# Autodesk Inventor assembly: V3IntakeNEW
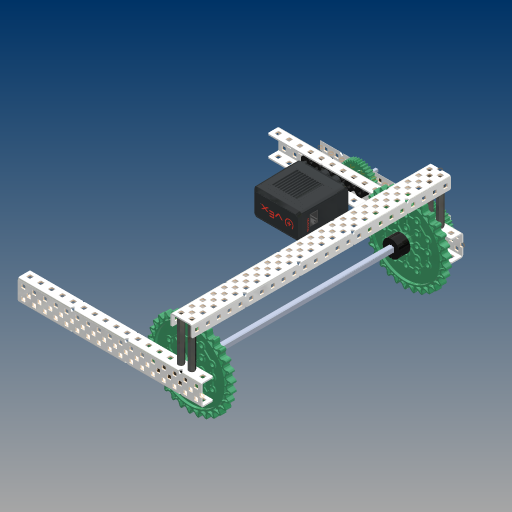
[picture p0: Inventor's stored thumbnail of the model, 512x512]
Saved by Autodesk Inventor 2024 (Build 280153000, 153)
## iProperties
Created: 2023-09-16
Part Number: V3IntakeNEW
Document SubType Name: Assembly
Designer: eddie
Author: eddie
## Documents named in this file (18)
- C:\Users\eddie\Documents\81208X-Over-Under-CAD\V3\V3IntakeNEW.iam
- C:\Users\eddie\Documents\81208X-Over-Under-CAD\VEX-CAD-Inventor-1.4.0\Structure\C Channel\Aluminum 1x2x1\Alu C 1x2x1x17.ipt
- C:\Users\eddie\Documents\81208X-Over-Under-CAD\VEX-CAD-Inventor-1.4.0\Structure\Standoff\Standoff 2.00.ipt
- C:\Users\eddie\Documents\81208X-Over-Under-CAD\VEX-CAD-Inventor-1.4.0\Structure\Standoff.ipt
- C:\Users\eddie\Documents\81208X-Over-Under-CAD\VEX-CAD-Inventor-1.4.0\Structure\C Channel\Aluminum 1x2x1\Alu C 1x2x1x24.ipt
- C:\Users\eddie\Documents\81208X-Over-Under-CAD\VEX-CAD-Inventor-1.4.0\Motion\Shaft LS\Bearing Flat.ipt
- C:\Users\eddie\Documents\81208X-Over-Under-CAD\VEX-CAD-Inventor-1.4.0\Motion\Spacers\Spacer Nylon .375 OD\NSpacer .375 OD x .500.ipt
- C:\Users\eddie\Documents\81208X-Over-Under-CAD\VEX-CAD-Inventor-1.4.0\Motion\Spacers\Spacer Nylon .375 OD.ipt
- C:\Users\eddie\Documents\81208X-Over-Under-CAD\VEX-CAD-Inventor-1.4.0\Motion\Shaft HS\Shaft HS\Shaft HS 12.0 in.ipt
- C:\Users\eddie\Documents\81208X-Over-Under-CAD\VEX-CAD-Inventor-1.4.0\Motion\Shaft HS\Shaft HS.ipt
- C:\Users\eddie\Documents\81208X-Over-Under-CAD\VEX-CAD-Inventor-1.4.0\Motion\Sprockets\9P Sprocket\9P 30T Sprocket, No Insert.iam
- C:\Users\eddie\Documents\81208X-Over-Under-CAD\VEX-CAD-Inventor-1.4.0\Motion\Sprockets\9P Sprocket.iam
- C:\Users\eddie\Documents\81208X-Over-Under-CAD\VEX-CAD-Inventor-1.4.0\Motion\Shaft HS\HS Shaft Collar.ipt
- C:\Users\eddie\Documents\81208X-Over-Under-CAD\VEX-CAD-Inventor-1.4.0\Motion\Gears\LS 36T Gear.ipt
- C:\Users\eddie\Documents\81208X-Over-Under-CAD\Custom-parts\2x12 c channel no sides.ipt
- C:\Users\eddie\Documents\81208X-Over-Under-CAD\VEX-CAD-Inventor-1.4.0\Motion\Shaft LS\Shaft LS.ipt
- C:\Users\eddie\Documents\81208X-Over-Under-CAD\VEX-CAD-Inventor-1.4.0\Motion\Shaft LS\Shaft LS\Shaft LS 1.0.ipt
- C:\Users\eddie\Documents\81208X-Over-Under-CAD\VEX-CAD-Inventor-1.4.0\Electronics\V5 Motor.ipt
## Components (24 placed, 12 different names)
1. Alu C 1x2x1x17:1 — Insert:1, Insert:2, Insert:7
2. Alu C 1x2x1x17:2 — Insert:4, Insert:5, Insert:10, Insert:16, Insert:21, Insert:22, Insert:23, Insert:24
3. Standoff 2.00:1 — Insert:2
4. Standoff 2.00:2 — Insert:1, Insert:3
5. Alu C 1x2x1x24:1 — Insert:3, Insert:6
6. Standoff 2.00:3 — Insert:5, Insert:6
7. Standoff 2.00:4 — Insert:4
8. Bearing Flat:1 — Insert:7, Insert:8, Insert:9
9. NSpacer .375 OD x .500:1 — Insert:8, Insert:12
10. Shaft HS 12.0 in:1 — Insert:9
11. Bearing Flat:2 — Insert:10, Insert:11
12. NSpacer .375 OD x .500:2 — Insert:11, Insert:13
13. 9P 30T Sprocket, No Insert:1 [sub-assembly] — Insert:12, Insert:14
14. 9P 30T Sprocket, No Insert:2 [sub-assembly] — Insert:13, Insert:26
15. HS Shaft Collar:1 — Insert:14
16. LS 36T Gear:1 — Insert:16, Insert:19
17. 2x12 c channel no sides:1 — Insert:19, Insert:20
18. Bearing Flat:3 — Insert:20
19. Shaft LS 1.0:1 — Insert:21
20. LS 36T Gear:2 — Insert:22
21. Bearing Flat:4 — Insert:23
22. Bearing Flat:5 — Insert:24, Insert:25
23. V5 Motor:1 — Insert:25
24. HS Shaft Collar:3 — Insert:26
## Relationships (23: Insert 23)
- Insert:1: Alu C 1x2x1x17:1 ↔ Standoff 2.00:2
- Insert:2: Alu C 1x2x1x17:1 ↔ Standoff 2.00:1
- Insert:3: Standoff 2.00:2 ↔ Alu C 1x2x1x24:1
- Insert:4: Alu C 1x2x1x17:2 ↔ Standoff 2.00:4
- Insert:5: Alu C 1x2x1x17:2 ↔ Standoff 2.00:3
- Insert:6: Alu C 1x2x1x24:1 ↔ Standoff 2.00:3
- Insert:7: Alu C 1x2x1x17:1 ↔ Bearing Flat:1
- Insert:8: Bearing Flat:1 ↔ NSpacer .375 OD x .500:1
- Insert:9: Bearing Flat:1 ↔ Shaft HS 12.0 in:1
- Insert:10: Alu C 1x2x1x17:2 ↔ Bearing Flat:2
- Insert:11: Bearing Flat:2 ↔ NSpacer .375 OD x .500:2
- Insert:12: NSpacer .375 OD x .500:1 ↔ 9P 30T Sprocket, No Insert:1
- Insert:13: NSpacer .375 OD x .500:2 ↔ 9P 30T Sprocket, No Insert:2
- Insert:14: 9P 30T Sprocket, No Insert:1 ↔ HS Shaft Collar:1
- Insert:16: Alu C 1x2x1x17:2 ↔ LS 36T Gear:1
- Insert:19: LS 36T Gear:1 ↔ 2x12 c channel no sides:1
- Insert:20: 2x12 c channel no sides:1 ↔ Bearing Flat:3
- Insert:21: Alu C 1x2x1x17:2 ↔ Shaft LS 1.0:1
- Insert:22: Alu C 1x2x1x17:2 ↔ LS 36T Gear:2
- Insert:23: Alu C 1x2x1x17:2 ↔ Bearing Flat:4
- Insert:24: Alu C 1x2x1x17:2 ↔ Bearing Flat:5
- Insert:25: Bearing Flat:5 ↔ V5 Motor:1
- Insert:26: 9P 30T Sprocket, No Insert:2 ↔ HS Shaft Collar:3
